# Autodesk Inventor assembly: leg_bone_2_MIR1
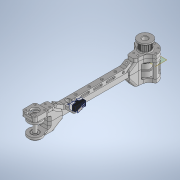
[picture p0: Inventor's stored thumbnail of the model, 180x180]
Saved by Autodesk Inventor 2020 (Build 240168000, 168)
## iProperties
Created: 2019-05-03
Part Number: leg_bone_2_MIR1
Document SubType Name: Assembly
Designer: psrob
Author: psrob
## Documents named in this file (13)
- E:\projects-2\project dog gen2\hardware\leg_bone_2_MIR1.iam
- E:\projects-2\project dog gen2\hardware\bone_upper_1_MIR.ipt
- E:\projects-2\project dog gen2\hardware\bone_upper_2_MIR.ipt
- E:\projects-2\project dog gen2\hardware\bone_upper_3_MIR.ipt
- E:\projects-2\project dog gen2\hardware\bone_upper_4_MIR.ipt
- E:\projects-2\project dog gen2\hardware\bearing_4_9_4_MIR.ipt
- E:\projects-2\project dog gen2\hardware\pin_2_20_MIR.ipt
- E:\projects-2\project dog gen2\hardware\bone_upper_wheel_1_MIR.ipt
- E:\projects-2\project dog gen2\hardware\2GT_wheel_MIR.ipt
- E:\projects-2\project dog gen2\hardware\carbon_fiber_70_MIR.ipt
- E:\projects-2\project dog gen2\hardware\leg_switch_holder_1_MIR.ipt
- E:\projects-2\project dog gen2\hardware\ultra-subminiature-basic-switch-d2f-1.snapshot.2\D2F-01L_MIR.ipt
- E:\projects-2\project dog gen2\hardware\encoder_holder_down_MIR.ipt
## Components (14 placed, 12 different names)
1. bone_upper_1_MIR:1 — Insert:2, Insert:1, Insert:8, Mate:5, Mate:4
2. bone_upper_1_MIR:2 — Insert:2, Insert:1, Insert:7, Mate:6, Insert:14, Insert:17, Insert:18
3. bone_upper_2_MIR:1 — Insert:4, Insert:3, Insert:6, Insert:11, Insert:10, Mate:3, Mate:1, Insert:13
4. bone_upper_3_MIR:1 — Insert:4, Insert:3, Insert:5, Flush:2, Insert:12, Mate:2
5. bone_upper_4_MIR:1 — Insert:6, Insert:5, Flush:2
6. bearing_4_9_4_MIR:1 — Insert:7, Insert:9
7. bearing_4_9_4_MIR:2 — Insert:8
8. pin_2_20_MIR:1 — Insert:9
9. bone_upper_wheel_1_MIR:1 — Insert:11, Insert:10
10. 2GT_wheel_MIR:1 — Insert:12
11. carbon_fiber_70_MIR:1 — Mate:6, Mate:5, Mate:4, Mate:3, Mate:2, Mate:1, Flush:3
12. leg_switch_holder_1_MIR:1 — Insert:14, Insert:13, Flush:3, Insert:16, Insert:15
13. D2F-01L_MIR:1 — Insert:16, Insert:15
14. encoder_holder_down_MIR:1 — Insert:17, Insert:18
## Relationships (26: Insert 18, Mate 8)
- Insert:2: bone_upper_1_MIR:1 ↔ bone_upper_1_MIR:2
- Insert:1: bone_upper_1_MIR:1 ↔ bone_upper_1_MIR:2
- Insert:4: bone_upper_2_MIR:1 ↔ bone_upper_3_MIR:1
- Insert:3: bone_upper_2_MIR:1 ↔ bone_upper_3_MIR:1
- Insert:6: bone_upper_2_MIR:1 ↔ bone_upper_4_MIR:1
- Insert:5: bone_upper_3_MIR:1 ↔ bone_upper_4_MIR:1
- Flush:2 [Mate]: bone_upper_3_MIR:1 ↔ bone_upper_4_MIR:1
- Insert:7: bone_upper_1_MIR:2 ↔ bearing_4_9_4_MIR:1
- Insert:8: bone_upper_1_MIR:1 ↔ bearing_4_9_4_MIR:2
- Insert:9 (0.5 mm): bearing_4_9_4_MIR:1 ↔ pin_2_20_MIR:1
- Insert:11: bone_upper_2_MIR:1 ↔ bone_upper_wheel_1_MIR:1
- Insert:10: bone_upper_2_MIR:1 ↔ bone_upper_wheel_1_MIR:1
- Insert:12 (0.3 mm): bone_upper_3_MIR:1 ↔ 2GT_wheel_MIR:1
- Mate:6: bone_upper_1_MIR:2 ↔ carbon_fiber_70_MIR:1
- Mate:5: bone_upper_1_MIR:1 ↔ carbon_fiber_70_MIR:1
- Mate:4: bone_upper_1_MIR:1 ↔ carbon_fiber_70_MIR:1
- Mate:3: bone_upper_2_MIR:1 ↔ carbon_fiber_70_MIR:1
- Mate:2: bone_upper_3_MIR:1 ↔ carbon_fiber_70_MIR:1
- Mate:1: bone_upper_2_MIR:1 ↔ carbon_fiber_70_MIR:1
- Insert:14: bone_upper_1_MIR:2 ↔ leg_switch_holder_1_MIR:1
- Insert:13: bone_upper_2_MIR:1 ↔ leg_switch_holder_1_MIR:1
- Flush:3 [Mate]: carbon_fiber_70_MIR:1 ↔ leg_switch_holder_1_MIR:1
- Insert:16: leg_switch_holder_1_MIR:1 ↔ D2F-01L_MIR:1
- Insert:15: leg_switch_holder_1_MIR:1 ↔ D2F-01L_MIR:1
- Insert:17: bone_upper_1_MIR:2 ↔ encoder_holder_down_MIR:1
- Insert:18: bone_upper_1_MIR:2 ↔ encoder_holder_down_MIR:1
